# Autodesk Inventor assembly: 240621_조립1
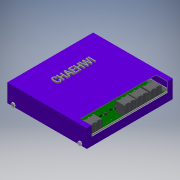
[picture p0: Inventor's stored thumbnail of the model, 180x180]
Saved by Autodesk Inventor 2016 (Build 200138000, 138)
## iProperties
Created: 2024-06-21
Part Number: 240621_조립1
Material: 일반
Document SubType Name: Assembly
Designer: pc
Author: pc
## Documents named in this file (6)
- D:\CAD_HCH\240621\240621_조립1.iam
- D:\CAD_HCH\240621\SCRAP CHIP V1.0.iam
- D:\CAD_HCH\240621\240621_pt1.ipt
- D:\CAD_HCH\240621\240621_나사.ipt
- D:\CAD_HCH\240621\240621_뚜껑.ipt
- C:\Users\pc\Documents\Inventor\Content Center Files\R2016\ko-KR\GB 5784-86\Bolt GB 5784-86-M3 x 20.ipt
## Components (11 placed, 5 different names)
1. SCRAP CHIP V1.0:1 [sub-assembly] — 메이트:1, 메이트:2, 메이트:3
2. 240621_pt1:1 — 메이트:1, 메이트:2, 메이트:3, 메이트:4, 플러쉬:1, 메이트:5, 플러쉬:2, 메이트:6, 플러쉬:3, 메이트:7, 플러쉬:4, 메이트:8, 메이트:9
3. 240621_나사:1 — 메이트:4, 플러쉬:1
4. 240621_나사:2 — 메이트:6, 플러쉬:3
5. 240621_나사:3 — 메이트:7, 플러쉬:4
6. 240621_나사:4 — 메이트:5, 플러쉬:2
7. 240621_뚜껑:1 — 메이트:8, 메이트:9, 삽입:1, 삽입:2, 삽입:3, 삽입:4
8. Bolt GB/T 5784-1986 M3x20:1 — 삽입:1
9. Bolt GB/T 5784-1986 M3x20:2 — 삽입:2
10. Bolt GB/T 5784-1986 M3x20:3 — 삽입:3
11. Bolt GB/T 5784-1986 M3x20:4 — 삽입:4
## Relationships (17: Mate 9, Flush 4, Insert 4)
- 메이트:1 [Mate] (4.8 mm): SCRAP CHIP V1.0:1 ↔ 240621_pt1:1
- 메이트:2 [Mate] (1 mm): SCRAP CHIP V1.0:1 ↔ 240621_pt1:1
- 메이트:3 [Mate] (1 mm): SCRAP CHIP V1.0:1 ↔ 240621_pt1:1
- 메이트:4 [Mate]: 240621_pt1:1 ↔ 240621_나사:1
- 플러쉬:1 [Flush]: 240621_pt1:1 ↔ 240621_나사:1
- 메이트:5 [Mate]: 240621_pt1:1 ↔ 240621_나사:4
- 플러쉬:2 [Flush]: 240621_pt1:1 ↔ 240621_나사:4
- 메이트:6 [Mate]: 240621_pt1:1 ↔ 240621_나사:2
- 플러쉬:3 [Flush]: 240621_pt1:1 ↔ 240621_나사:2
- 메이트:7 [Mate]: 240621_pt1:1 ↔ 240621_나사:3
- 플러쉬:4 [Flush]: 240621_pt1:1 ↔ 240621_나사:3
- 메이트:8 [Mate]: 240621_pt1:1 ↔ 240621_뚜껑:1
- 메이트:9 [Mate]: 240621_pt1:1 ↔ 240621_뚜껑:1
- 삽입:1 [Insert]: 240621_뚜껑:1 ↔ Bolt GB/T 5784-1986 M3x20:1
- 삽입:2 [Insert]: 240621_뚜껑:1 ↔ Bolt GB/T 5784-1986 M3x20:2
- 삽입:3 [Insert]: 240621_뚜껑:1 ↔ Bolt GB/T 5784-1986 M3x20:3
- 삽입:4 [Insert]: 240621_뚜껑:1 ↔ Bolt GB/T 5784-1986 M3x20:4
